# Autodesk Inventor assembly: SCS8UU
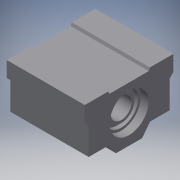
[picture p0: Inventor's stored thumbnail of the model, 180x180]
Saved by Autodesk Inventor 2018 (Build 220112000, 112)
## iProperties
Created: 2018-09-20
Part Number: SCS8UU
Material: Genérico
Document SubType Name: Assembly
Designer: Georgines
Author: Georgines
## Documents named in this file (4)
- C:\Users\Georgines\Documents\EstacaoBGA\Peças 3D\SCS8UU.iam
- C:\Users\Georgines\Documents\EstacaoBGA\Peças 3D\rolamento_linear_lm8uu.iam.ipt
- C:\Users\Georgines\Documents\EstacaoBGA\Peças 3D\PilowBlockFechadoSCS8UU.ipt
- rolamento_linear_lm8uu.iam
## Components (2 placed, 2 different names)
1. rolamento_linear_lm8uu.iam:1 — Coincidência:1, Alinhamento:1
2. PilowBlockFechadoSCS8UU:1 — Coincidência:1, Alinhamento:1
## Relationships (2: Mate 1, Flush 1)
- Coincidência:1 [Mate]: rolamento_linear_lm8uu.iam:1 ↔ PilowBlockFechadoSCS8UU:1
- Alinhamento:1 [Flush] (3 mm): rolamento_linear_lm8uu.iam:1 ↔ PilowBlockFechadoSCS8UU:1
